# Autodesk Inventor assembly: TomatoArm1
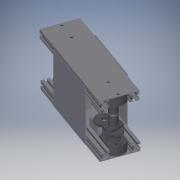
[picture p0: Inventor's stored thumbnail of the model, 180x180]
Saved by Autodesk Inventor 2016 (Build 200138000, 138)
## iProperties
Created: 2016-06-28
Part Number: TomatoArm1
Material: 一般
Document SubType Name: Assembly
Designer: 宏太
Author: 宏太
## Documents named in this file (10)
- C:\Users\宏太\Documents\Inventor\Content Center Files\Tomoto2016\TomatoArm1.iam
- C:\Users\宏太\Documents\Inventor\Content Center Files\Tomoto2016\NFS5-2020-260.ipt
- C:\Users\宏太\Documents\Inventor\Content Center Files\Tomoto2016\BGCSB9\BGCSB9.iam
- C:\Users\宏太\Documents\Inventor\Content Center Files\Tomoto2016\bottom_board.ipt
- C:\Users\宏太\Documents\Inventor\Content Center Files\Tomoto2016\shaft2016.ipt
- C:\Users\宏太\Documents\Inventor\Content Center Files\Tomoto2016\GEAHBB1.0-40-6-A-12\GEAHBB1_0-40-6-A-12.iam
- C:\Users\宏太\Documents\Inventor\Content Center Files\Tomoto2016\GEAHBB1.0-40-6-B-12\GEAHBB1_0-40-6-B-12.iam
- C:\Users\宏太\Documents\Inventor\Content Center Files\Tomoto2016\STHCBT15-MB\STHCBT15-MB.iam
- C:\Users\宏太\Documents\Inventor\Content Center Files\Tomoto2016\Servo.iam
- C:\Users\宏太\Documents\Inventor\Content Center Files\Tomoto2016\Side_board.ipt
## Components (24 placed, 9 different names)
1. NFS5-2020-260:2 — フラッシュ:12, フラッシュ:13, メイト:6
2. NFS5-2020-260:4 — フラッシュ:10, フラッシュ:11
3. NFS5-2020-260:5 — フラッシュ:17, メイト:7, フラッシュ:18, メイト:11
4. NFS5-2020-260:6 — フラッシュ:14, フラッシュ:15, フラッシュ:16, メイト:13
5. BGCSB9:1 [sub-assembly] — 挿入:9, 挿入:12, 挿入:14
6. BGCSB9:2 [sub-assembly] — 挿入:10, 挿入:11, 挿入:13
7. bottom_board:1 — フラッシュ:9, 挿入:9, 挿入:10, 挿入:11, フラッシュ:10, フラッシュ:11, フラッシュ:12, フラッシュ:13, メイト:6, 挿入:14, メイト:12
8. shaft2016:1 — 挿入:12, 挿入:15, 挿入:16, 挿入:20, 挿入:21
9. shaft2016:2 — 挿入:13, 挿入:17, 挿入:18, 挿入:19, 挿入:22
10. GEAHBB1_0-40-6-A-12:1 [sub-assembly] — 挿入:26
11. GEAHBB1_0-40-6-A-12:2 [sub-assembly] — 挿入:27
12. GEAHBB1_0-40-6-B-12:1 [sub-assembly] — 挿入:22
13. GEAHBB1_0-40-6-B-12:2 [sub-assembly] — 挿入:21
14. BGCSB9:3 [sub-assembly] — 挿入:19, 挿入:23, 挿入:24
15. BGCSB9:4 [sub-assembly] — 挿入:20, 挿入:25
16. bottom_board:2 — 挿入:23, 挿入:24, 挿入:25, フラッシュ:14, フラッシュ:15, フラッシュ:16, フラッシュ:17, メイト:7, フラッシュ:18, メイト:8, フラッシュ:19, フラッシュ:20, メイト:9, フラッシュ:21, フラッシュ:22, メイト:10, フラッシュ:23, フラッシュ:24
17. STHCBT15-MB:1 [sub-assembly] — 挿入:16
18. STHCBT15-MB:2 [sub-assembly] — 挿入:18
19. STHCBT15-MB:3 [sub-assembly] — 挿入:17
20. STHCBT15-MB:4 [sub-assembly] — 挿入:15
21. Servo:1 [sub-assembly] — メイト:9, フラッシュ:21, 挿入:26, フラッシュ:22
22. Servo:2 [sub-assembly] — メイト:8, フラッシュ:19, フラッシュ:20, 挿入:27
23. Side_board:1 — メイト:10, フラッシュ:23, メイト:11
24. Side_board:2 — フラッシュ:24, メイト:12, メイト:13
## Relationships (43: Insert 19, Flush 16, Mate 8)
- フラッシュ:9 [Flush]: bottom_board:1
- 挿入:9 [Insert]: BGCSB9:1 ↔ bottom_board:1
- 挿入:10 [Insert]: BGCSB9:2 ↔ bottom_board:1
- 挿入:11 [Insert]: BGCSB9:2 ↔ bottom_board:1
- フラッシュ:10 [Flush]: NFS5-2020-260:4 ↔ bottom_board:1
- フラッシュ:11 [Flush]: NFS5-2020-260:4 ↔ bottom_board:1
- フラッシュ:12 [Flush]: NFS5-2020-260:2 ↔ bottom_board:1
- フラッシュ:13 [Flush]: NFS5-2020-260:2 ↔ bottom_board:1
- 挿入:12 [Insert]: BGCSB9:1 ↔ shaft2016:1
- 挿入:13 [Insert]: BGCSB9:2 ↔ shaft2016:2
- メイト:6 [Mate]: NFS5-2020-260:2 ↔ bottom_board:1
- 挿入:14 [Insert]: BGCSB9:1 ↔ bottom_board:1
- 挿入:15 [Insert] (60 mm): shaft2016:1 ↔ STHCBT15-MB:4
- 挿入:16 [Insert] (-55 mm): shaft2016:1 ↔ STHCBT15-MB:1
- 挿入:17 [Insert] (60 mm): shaft2016:2 ↔ STHCBT15-MB:3
- 挿入:18 [Insert] (-55 mm): shaft2016:2 ↔ STHCBT15-MB:2
- 挿入:19 [Insert]: shaft2016:2 ↔ BGCSB9:3
- 挿入:20 [Insert]: shaft2016:1 ↔ BGCSB9:4
- 挿入:21 [Insert] (-20 mm): shaft2016:1 ↔ GEAHBB1_0-40-6-B-12:2
- 挿入:22 [Insert] (-20 mm): shaft2016:2 ↔ GEAHBB1_0-40-6-B-12:1
- 挿入:23 [Insert]: BGCSB9:3 ↔ bottom_board:2
- 挿入:24 [Insert]: BGCSB9:3 ↔ bottom_board:2
- 挿入:25 [Insert]: BGCSB9:4 ↔ bottom_board:2
- フラッシュ:14 [Flush]: NFS5-2020-260:6 ↔ bottom_board:2
- フラッシュ:15 [Flush]: NFS5-2020-260:6 ↔ bottom_board:2
- フラッシュ:16 [Flush] (2 mm): NFS5-2020-260:6 ↔ bottom_board:2
- フラッシュ:17 [Flush]: NFS5-2020-260:5 ↔ bottom_board:2
- メイト:7 [Mate]: NFS5-2020-260:5 ↔ bottom_board:2
- フラッシュ:18 [Flush]: NFS5-2020-260:5 ↔ bottom_board:2
- メイト:8 [Mate]: bottom_board:2 ↔ Servo:2
- フラッシュ:19 [Flush] (162 mm): bottom_board:2 ↔ Servo:2
- フラッシュ:20 [Flush] (25 mm): bottom_board:2 ↔ Servo:2
- メイト:9 [Mate]: bottom_board:2 ↔ Servo:1
- フラッシュ:21 [Flush] (162 mm): bottom_board:2 ↔ Servo:1
- 挿入:26 [Insert]: GEAHBB1_0-40-6-A-12:1 ↔ Servo:1
- 挿入:27 [Insert]: GEAHBB1_0-40-6-A-12:2 ↔ Servo:2
- フラッシュ:22 [Flush] (25 mm): bottom_board:2 ↔ Servo:1
- メイト:10 [Mate]: bottom_board:2 ↔ Side_board:1
- フラッシュ:23 [Flush] (60 mm): bottom_board:2 ↔ Side_board:1
- メイト:11 [Mate]: NFS5-2020-260:5 ↔ Side_board:1
- フラッシュ:24 [Flush] (60 mm): bottom_board:2 ↔ Side_board:2
- メイト:12 [Mate]: bottom_board:1 ↔ Side_board:2
- メイト:13 [Mate]: NFS5-2020-260:6 ↔ Side_board:2
